# Autodesk Inventor assembly: bottom_hinge_pot
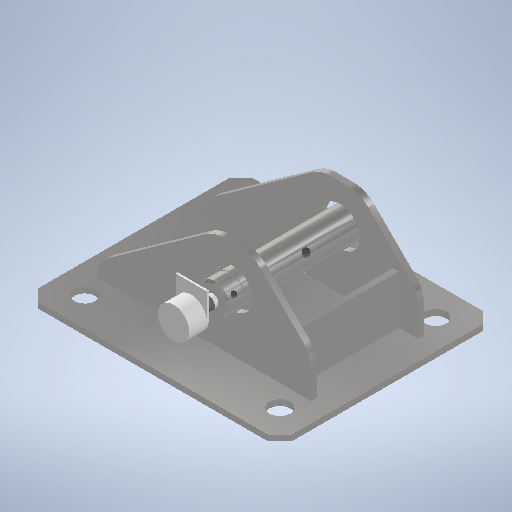
[picture p0: Inventor's stored thumbnail of the model, 512x512]
Saved by Autodesk Inventor 2025.2 (Build 292293000, 293)
## iProperties
Created: 2025-03-24
Part Number: bottom_hinge_pot
Document SubType Name: Assembly
Designer: Caspe
Author: Caspe
## Documents named in this file (6)
- C:\Users\Caspe\Documents\Semester 8\Project\Anomaly_Detection\Mechanical_Project\Inventor_project\bottom_hinge_pot.iam
- C:\Users\Caspe\Documents\Semester 8\Project\Anomaly_Detection\Mechanical_Project\Inventor_project\bottom_hinge_001.ipt
- C:\Users\Caspe\Documents\Semester 8\Project\Anomaly_Detection\Mechanical_Project\Inventor_project\bottom_hinge_002.ipt
- C:\Users\Caspe\Documents\Semester 8\Project\Anomaly_Detection\Mechanical_Project\Inventor_project\bottom_hinge_003.ipt
- C:\Users\Caspe\Documents\Semester 8\Project\Anomaly_Detection\Mechanical_Project\Inventor_project\shaft potmeter.ipt
- C:\Users\Caspe\Documents\Semester 8\Project\Anomaly_Detection\Mechanical_Project\Inventor_project\Potentiometer.ipt
## Components (6 placed, 5 different names)
1. bottom_hinge_001:1 — Mate:1, Mate:2, Mate:4, Mate:6
2. bottom_hinge_002:1 — Mate:1, Mate:2, Mate:5, Mate:7
3. bottom_hinge_003:1 — Mate:4, Mate:5, Mate:8
4. bottom_hinge_003:2 — Mate:6, Mate:7, Flush:1
5. shaft potmeter:1 — Mate:8, Flush:1, Mate:9, Mate:10
6. Potentiometer:1 — Mate:9, Mate:10
## Relationships (10: Mate 9, Flush 1)
- Mate:1: bottom_hinge_001:1 ↔ bottom_hinge_002:1
- Mate:2: bottom_hinge_001:1 ↔ bottom_hinge_002:1
- Mate:4: bottom_hinge_001:1 ↔ bottom_hinge_003:1
- Mate:5: bottom_hinge_002:1 ↔ bottom_hinge_003:1
- Mate:6: bottom_hinge_001:1 ↔ bottom_hinge_003:2
- Mate:7: bottom_hinge_002:1 ↔ bottom_hinge_003:2
- Mate:8: bottom_hinge_003:1 ↔ shaft potmeter:1
- Flush:1 (-10.5 mm): bottom_hinge_003:2 ↔ shaft potmeter:1
- Mate:9: shaft potmeter:1 ↔ Potentiometer:1
- Mate:10: shaft potmeter:1 ↔ Potentiometer:1
